# Autodesk Inventor assembly: Cube 1x1 V5 (Half Inch Lense)
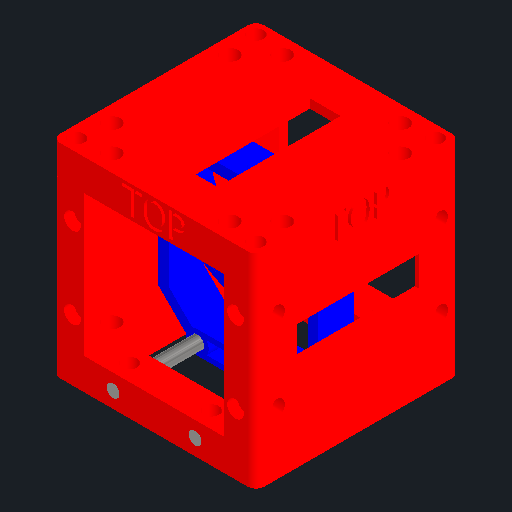
[picture p0: Inventor's stored thumbnail of the model, 512x512]
Saved by Autodesk Inventor 2023.4 (Build 274418000, 418)
## iProperties
Created: 2022-08-13
Part Number: Cube 1x1 V5 (Half Inch Lense)
Document SubType Name: Assembly
Designer: xSibe
Author: xSibe
## Documents named in this file (5)
- C:\.Laptop\.Work\Projects\Project Protocube\1 Autodesk\1 Cubes\Lense\Cube 1x1 V5 (Half Inch Lense).iam
- C:\.Laptop\.Work\Projects\Project Protocube\1 Autodesk\1 Cubes\Attachments\Mounting Bar.ipt
- C:\.Laptop\.Work\Projects\Project Protocube\1 Autodesk\1 Cubes\Lense\Half Inch Lense Holder (V5).ipt
- C:\.Laptop\.Work\Projects\Project Protocube\1 Autodesk\1 Cubes\Cubes\Cube 1x1 V5 Closed Slotted.iam
- C:\.Laptop\.Work\Projects\Project Protocube\1 Autodesk\1 Cubes\Lense\Half Inch Lense Holder Cover (V5).ipt
## Components (4 placed, 4 different names)
1. Mounting Bar:1
2. Half Inch Lense Holder (V5):1 — Mate:1, Mate:2
3. Cube 1x1 V5 Closed Slotted:1 [sub-assembly]
4. Half Inch Lense Holder Cover (V5):1 — Mate:1, Mate:2, Flush:1
## Relationships (3: Mate 2, Flush 1)
- Mate:1: Half Inch Lense Holder (V5):1 ↔ Half Inch Lense Holder Cover (V5):1
- Mate:2: Half Inch Lense Holder (V5):1 ↔ Half Inch Lense Holder Cover (V5):1
- Flush:1: Half Inch Lense Holder Cover (V5):1
